# Autodesk Inventor assembly: main
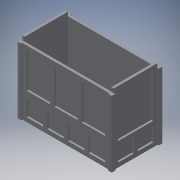
[picture p0: Inventor's stored thumbnail of the model, 180x180]
Saved by Autodesk Inventor 2017 (Build 210142000, 142)
## iProperties
Created: 2019-05-05
Part Number: main
Document SubType Name: Assembly
Designer: Roman
Author: Roman
## Documents named in this file (5)
- C:\Users\Roman\Documents\CAD\tegu rev2\main.iam
- C:\Users\Roman\Documents\CAD\tegu rev2\base\base.iam
- C:\Users\Roman\Documents\CAD\tegu rev2\floor\floor.iam
- C:\Users\Roman\Documents\CAD\tegu rev2\upper walls\long wall\upper long wall.iam
- C:\Users\Roman\Documents\CAD\tegu rev2\upper walls\short wall\short wall.iam
## Components (6 placed, 4 different names)
1. base:1 [sub-assembly] — Flush:1, Mate:1, Mate:2, Flush:2, Mate:3, Mate:4, Flush:3, Mate:5, Mate:6, Flush:4, Flush:5
2. floor:1 [sub-assembly] — Flush:1, Mate:1, Mate:2
3. upper long wall:1 [sub-assembly] — Flush:2, Mate:3, Mate:4
4. upper long wall:2 [sub-assembly] — Flush:3, Mate:5, Mate:6
5. short wall:1 [sub-assembly] — Flush:5
6. short wall:2 [sub-assembly] — Flush:4
## Relationships (11: Mate 6, Flush 5)
- Flush:1: base:1 ↔ floor:1
- Mate:1: base:1 ↔ floor:1
- Mate:2: base:1 ↔ floor:1
- Flush:2: base:1 ↔ upper long wall:1
- Mate:3: base:1 ↔ upper long wall:1
- Mate:4: base:1 ↔ upper long wall:1
- Flush:3: base:1 ↔ upper long wall:2
- Mate:5: base:1 ↔ upper long wall:2
- Mate:6: base:1 ↔ upper long wall:2
- Flush:4: base:1 ↔ short wall:2
- Flush:5: base:1 ↔ short wall:1
